# Autodesk Inventor assembly: 조립품2
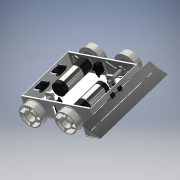
[picture p0: Inventor's stored thumbnail of the model, 180x180]
Saved by Autodesk Inventor 2017 (Build 210142000, 142)
## iProperties
Part Number: 조립품2
Material: 일반
Document SubType Name: Assembly
Designer: minom
Author: minom
## Documents named in this file (19)
- C:\Users\minom\Documents\Inventor\Projects\2017 IRC Sumo Mino\조립품2.iam
- C:\Users\minom\Documents\Inventor\Projects\2017 IRC Sumo Mino\옆판.ipt
- C:\Users\minom\Documents\Inventor\Projects\2017 IRC Sumo Mino\밑판.ipt
- C:\Users\minom\Documents\Inventor\Projects\2017 IRC Sumo Mino\뒷판.ipt
- C:\Users\minom\Documents\Inventor\Projects\2017 IRC Sumo Mino\앞판_밑.ipt
- C:\Users\minom\Documents\Inventor\Projects\2017 IRC Sumo Mino\앞판_중간.ipt
- C:\Users\minom\Documents\Inventor\Projects\2017 IRC Sumo Mino\앞판_위.ipt
- C:\Users\minom\Documents\Inventor\Projects\2017 IRC Sumo Mino\옆판_왼쪽.ipt
- C:\Users\minom\Documents\Inventor\Projects\영준이형 씨름로봇\IG-42GM_motor.ipt
- C:\Users\minom\Documents\Inventor\Projects\2017 IRC Sumo Mino\베어링받침대.ipt
- C:\Users\minom\Documents\Inventor\Projects\2017 IRC Sumo Mino\ATP25XL025-A-N10-KC90-QFC20-M3-FC45_0-TPC3.iam
- C:\Users\minom\Documents\Inventor\Projects\2017 IRC Sumo Mino\FL6700ZZ.ipt
- C:\Users\minom\Documents\Inventor\Projects\2017 IRC Sumo Mino\10PI축.ipt
- C:\Users\minom\Documents\Inventor\Projects\2017 IRC Sumo Mino\ATP25XL025-A-N8-KC90-QFC20-M3-FC45_0-TPC3.iam
- C:\Users\minom\Documents\Inventor\Projects\2017 IRC Sumo Mino\바퀴.ipt
- C:\Users\minom\Documents\Inventor\Projects\2017 IRC Sumo Mino\바퀴8PI.ipt
- C:\Users\minom\Documents\Inventor\Projects\영준이형 씨름로봇\PSD_2.ipt
- C:\Users\minom\Documents\Inventor\Projects\2017 IRC Sumo Mino\앞판바깥막이.ipt
- C:\Users\minom\Documents\Inventor\Projects\2017 IRC Sumo Mino\서포터 20.ipt
## Components (37 placed, 18 different names)
1. 옆판_오른쪽:1 — 메이트:4, 메이트:9, 플러쉬:7, 메이트:22, 메이트:23, 메이트:47, 메이트:50, 메이트:55, 플러쉬:19, 메이트:76
2. 밑판:1 — 메이트:4, 플러쉬:6, 메이트:12, 플러쉬:9, 메이트:21, 메이트:43, 메이트:44, 메이트:48, 메이트:49, 메이트:76, 메이트:83, 메이트:86, 메이트:87
3. 뒷판:1 — 플러쉬:6, 메이트:9, 플러쉬:7, 메이트:13, 메이트:89, 메이트:90, 메이트:93, 메이트:94
4. 앞판_밑:1 — 메이트:18, 메이트:80, 메이트:81, 메이트:85, 메이트:88
5. 앞판_중간:1 — 메이트:77, 메이트:78, 메이트:82, 메이트:84
6. 앞판_위:1 — 메이트:14, 메이트:19, 플러쉬:8
7. 옆판_왼쪽:1 — 메이트:12, 메이트:13, 메이트:14, 메이트:18, 메이트:19, 플러쉬:8, 플러쉬:9, 메이트:21, 메이트:24, 메이트:25, 메이트:42, 메이트:53, 메이트:57, 플러쉬:14, 메이트:77, 메이트:78, 메이트:80, 메이트:81, 메이트:82
8. IG-42GM_motor:1 — 메이트:22, 메이트:23, 메이트:65, 플러쉬:18, 메이트:72
9. IG-42GM_motor:2 — 메이트:24, 메이트:25, 메이트:64, 플러쉬:16, 메이트:70
10. 베어링받침대:1 — 메이트:42, 메이트:43, 메이트:44, 메이트:52, 메이트:56
11. 베어링받침대:2 — 메이트:47, 메이트:48, 메이트:49, 메이트:51, 메이트:54
12. ATP25XL025-A-N10-KC90-QFC20-M3-FC45_0-TPC3:1 [sub-assembly] — 메이트:61, 플러쉬:17, 메이트:67
13. ATP25XL025-A-N10-KC90-QFC20-M3-FC45_0-TPC3:2 [sub-assembly] — 메이트:62, 플러쉬:15, 메이트:74
14. FL6700ZZ:1 — 메이트:52, 메이트:56
15. FL6700ZZ:2 — 메이트:53, 메이트:57, 메이트:60
16. FL6700ZZ:3 — 메이트:51, 메이트:54
17. FL6700ZZ:4 — 메이트:50, 메이트:55, 메이트:58
18. 10PI축:1 — 메이트:58, 메이트:61, 플러쉬:19, 메이트:66
19. 10PI축:2 — 메이트:60, 플러쉬:14, 메이트:62, 메이트:68
20. ATP25XL025-A-N8-KC90-QFC20-M3-FC45_0-TPC3:1 [sub-assembly] — 메이트:64, 플러쉬:15, 플러쉬:16, 메이트:75
21. ATP25XL025-A-N8-KC90-QFC20-M3-FC45_0-TPC3:2 [sub-assembly] — 메이트:65, 플러쉬:17, 플러쉬:18, 메이트:73
22. 바퀴10PI:1 — 메이트:66, 메이트:67
23. 바퀴10PI:2 — 메이트:68, 메이트:74
24. 바퀴8PI:1 — 메이트:70, 메이트:75
25. 바퀴8PI:2 — 메이트:72, 메이트:73
26. PSD_2:1
27. PSD_2:2
28. PSD_2:3 — 메이트:91, 메이트:92, 메이트:97
29. PSD_2:4 — 메이트:95, 메이트:96, 메이트:98
30. 앞판바깥막이:1 — 메이트:83, 메이트:84, 메이트:85
31. 앞판바깥막이:2 — 메이트:86, 메이트:87, 메이트:88
32. PSD_2:5
33. PSD_2:6
34. 서포터 20:1 — 메이트:90, 메이트:92
35. 서포터 20:2 — 메이트:89, 메이트:91, 메이트:97
36. 서포터 20:3 — 메이트:94, 메이트:96
37. 서포터 20:4 — 메이트:93, 메이트:95, 메이트:98
## Relationships (72: Mate 62, Flush 10)
- 메이트:4 [Mate] (0.2 mm): 옆판_오른쪽:1 ↔ 밑판:1
- 플러쉬:6 [Flush]: 밑판:1 ↔ 뒷판:1
- 메이트:9 [Mate]: 옆판_오른쪽:1 ↔ 뒷판:1
- 플러쉬:7 [Flush]: 옆판_오른쪽:1 ↔ 뒷판:1
- 메이트:12 [Mate]: 밑판:1 ↔ 옆판_왼쪽:1
- 메이트:13 [Mate]: 뒷판:1 ↔ 옆판_왼쪽:1
- 메이트:14 [Mate] (0.2 mm): 앞판_위:1 ↔ 옆판_왼쪽:1
- 메이트:18 [Mate] (0.2 mm): 앞판_밑:1 ↔ 옆판_왼쪽:1
- 메이트:19 [Mate]: 앞판_위:1 ↔ 옆판_왼쪽:1
- 플러쉬:8 [Flush]: 앞판_위:1 ↔ 옆판_왼쪽:1
- 플러쉬:9 [Flush]: 밑판:1 ↔ 옆판_왼쪽:1
- 메이트:21 [Mate] (0.2 mm): 밑판:1 ↔ 옆판_왼쪽:1
- 메이트:22 [Mate]: 옆판_오른쪽:1 ↔ IG-42GM_motor:1
- 메이트:23 [Mate]: 옆판_오른쪽:1 ↔ IG-42GM_motor:1
- 메이트:24 [Mate]: 옆판_왼쪽:1 ↔ IG-42GM_motor:2
- 메이트:25 [Mate]: 옆판_왼쪽:1 ↔ IG-42GM_motor:2
- 메이트:42 [Mate] (40 mm): 옆판_왼쪽:1 ↔ 베어링받침대:1
- 메이트:43 [Mate]: 밑판:1 ↔ 베어링받침대:1
- 메이트:44 [Mate]: 밑판:1 ↔ 베어링받침대:1
- 메이트:47 [Mate] (40 mm): 옆판_오른쪽:1 ↔ 베어링받침대:2
- 메이트:48 [Mate]: 밑판:1 ↔ 베어링받침대:2
- 메이트:49 [Mate]: 밑판:1 ↔ 베어링받침대:2
- 메이트:50 [Mate]: 옆판_오른쪽:1 ↔ FL6700ZZ:4
- 메이트:51 [Mate]: 베어링받침대:2 ↔ FL6700ZZ:3
- 메이트:52 [Mate]: 베어링받침대:1 ↔ FL6700ZZ:1
- 메이트:53 [Mate]: 옆판_왼쪽:1 ↔ FL6700ZZ:2
- 메이트:54 [Mate]: 베어링받침대:2 ↔ FL6700ZZ:3
- 메이트:55 [Mate]: 옆판_오른쪽:1 ↔ FL6700ZZ:4
- 메이트:56 [Mate]: 베어링받침대:1 ↔ FL6700ZZ:1
- 메이트:57 [Mate]: 옆판_왼쪽:1 ↔ FL6700ZZ:2
- 메이트:58 [Mate]: FL6700ZZ:4 ↔ 10PI축:1
- 메이트:60 [Mate]: FL6700ZZ:2 ↔ 10PI축:2
- 플러쉬:14 [Flush] (-20 mm): 옆판_왼쪽:1 ↔ 10PI축:2
- 메이트:61 [Mate]: ATP25XL025-A-N10-KC90-QFC20-M3-FC45_0-TPC3:1 ↔ 10PI축:1
- 메이트:62 [Mate]: ATP25XL025-A-N10-KC90-QFC20-M3-FC45_0-TPC3:2 ↔ 10PI축:2
- 메이트:64 [Mate]: IG-42GM_motor:2 ↔ ATP25XL025-A-N8-KC90-QFC20-M3-FC45_0-TPC3:1
- 플러쉬:15 [Flush]: ATP25XL025-A-N10-KC90-QFC20-M3-FC45_0-TPC3:2 ↔ ATP25XL025-A-N8-KC90-QFC20-M3-FC45_0-TPC3:1
- 플러쉬:16 [Flush] (4 mm): IG-42GM_motor:2 ↔ ATP25XL025-A-N8-KC90-QFC20-M3-FC45_0-TPC3:1
- 메이트:65 [Mate]: IG-42GM_motor:1 ↔ ATP25XL025-A-N8-KC90-QFC20-M3-FC45_0-TPC3:2
- 플러쉬:17 [Flush]: ATP25XL025-A-N10-KC90-QFC20-M3-FC45_0-TPC3:1 ↔ ATP25XL025-A-N8-KC90-QFC20-M3-FC45_0-TPC3:2
- 플러쉬:18 [Flush] (4 mm): IG-42GM_motor:1 ↔ ATP25XL025-A-N8-KC90-QFC20-M3-FC45_0-TPC3:2
- 플러쉬:19 [Flush] (-20 mm): 옆판_오른쪽:1 ↔ 10PI축:1
- 메이트:66 [Mate]: 10PI축:1 ↔ 바퀴10PI:1
- 메이트:67 [Mate]: ATP25XL025-A-N10-KC90-QFC20-M3-FC45_0-TPC3:1 ↔ 바퀴10PI:1
- 메이트:68 [Mate]: 10PI축:2 ↔ 바퀴10PI:2
- 메이트:70 [Mate]: IG-42GM_motor:2 ↔ 바퀴8PI:1
- 메이트:72 [Mate]: IG-42GM_motor:1 ↔ 바퀴8PI:2
- 메이트:73 [Mate]: ATP25XL025-A-N8-KC90-QFC20-M3-FC45_0-TPC3:2 ↔ 바퀴8PI:2
- 메이트:74 [Mate]: ATP25XL025-A-N10-KC90-QFC20-M3-FC45_0-TPC3:2 ↔ 바퀴10PI:2
- 메이트:75 [Mate]: ATP25XL025-A-N8-KC90-QFC20-M3-FC45_0-TPC3:1 ↔ 바퀴8PI:1
- 메이트:76 [Mate]: 옆판_오른쪽:1 ↔ 밑판:1
- 메이트:77 [Mate]: 앞판_중간:1 ↔ 옆판_왼쪽:1
- 메이트:78 [Mate] (0.2 mm): 앞판_중간:1 ↔ 옆판_왼쪽:1
- 메이트:80 [Mate]: 앞판_밑:1 ↔ 옆판_왼쪽:1
- 메이트:81 [Mate]: 앞판_밑:1 ↔ 옆판_왼쪽:1
- 메이트:82 [Mate] (1 mm): 앞판_중간:1 ↔ 옆판_왼쪽:1
- 메이트:83 [Mate]: 밑판:1 ↔ 앞판바깥막이:1
- 메이트:84 [Mate]: 앞판_중간:1 ↔ 앞판바깥막이:1
- 메이트:85 [Mate] (0.2 mm): 앞판_밑:1 ↔ 앞판바깥막이:1
- 메이트:86 [Mate]: 밑판:1 ↔ 앞판바깥막이:2
- 메이트:87 [Mate] (0.2 mm): 밑판:1 ↔ 앞판바깥막이:2
- 메이트:88 [Mate]: 앞판_밑:1 ↔ 앞판바깥막이:2
- 메이트:89 [Mate]: 뒷판:1 ↔ 서포터 20:2
- 메이트:90 [Mate]: 뒷판:1 ↔ 서포터 20:1
- 메이트:91 [Mate]: PSD_2:3 ↔ 서포터 20:2
- 메이트:92 [Mate]: PSD_2:3 ↔ 서포터 20:1
- 메이트:93 [Mate]: 뒷판:1 ↔ 서포터 20:4
- 메이트:94 [Mate]: 뒷판:1 ↔ 서포터 20:3
- 메이트:95 [Mate]: PSD_2:4 ↔ 서포터 20:4
- 메이트:96 [Mate]: PSD_2:4 ↔ 서포터 20:3
- 메이트:97 [Mate] (1 mm): PSD_2:3 ↔ 서포터 20:2
- 메이트:98 [Mate] (1 mm): PSD_2:4 ↔ 서포터 20:4
